# Autodesk Inventor assembly: ControlBox
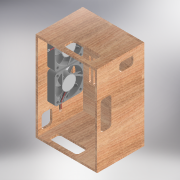
[picture p0: Inventor's stored thumbnail of the model, 180x180]
Saved by Autodesk Inventor 2018.2 (Build 222227000, 227)
## iProperties
Created: 2018-03-27
Part Number: ControlBox
Document SubType Name: Assembly
Designer: mansu
Author: mansu
## Documents named in this file (6)
- C:\Users\Moochster\OneDrive\Documents\2018 UBC\ELEC 391\Controller\cad\release\ControlBox.iam
- C:\Users\Moochster\OneDrive\Documents\2018 UBC\ELEC 391\Controller\cad\release\ControlBoxTop.ipt
- C:\Users\Moochster\OneDrive\Documents\2018 UBC\ELEC 391\Controller\cad\release\ControlBoxFace.ipt
- C:\Users\Moochster\OneDrive\Documents\2018 UBC\ELEC 391\Controller\cad\release\40x40x10 DC Fan.ipt
- C:\Users\Moochster\OneDrive\Documents\2018 UBC\ELEC 391\Controller\cad\release\ControlBoxFlatFace.ipt
- C:\Users\Moochster\OneDrive\Documents\2018 UBC\ELEC 391\Controller\cad\release\ControlBoxSide.ipt
## Components (7 placed, 5 different names)
1. ControlBoxTop:1 — Flush:5, Flush:6, Flush:8, Flush:9
2. ControlBoxFlatFace:1 — Flush:5, Mate:17, Mate:18, Mate:19, Mate:20, Flush:8
3. ControlBoxFace:2 — Flush:6, Mate:12, Mate:13, Mate:14, Mate:15, Mate:16, Mate:21, Mate:22
4. 40x40x10 DC Fan:1 — Mate:12, Flush:7, Mate:14, Mate:15
5. 40x40x10 DC Fan:2 — Mate:13, Flush:7, Mate:16
6. ControlBoxSide:1 — Mate:17, Mate:18, Mate:21, Mate:22, Flush:9
7. ControlBoxSide:2 — Mate:19, Mate:20
## Relationships (16: Mate 11, Flush 5)
- Flush:5: ControlBoxTop:1 ↔ ControlBoxFlatFace:1
- Flush:6: ControlBoxTop:1 ↔ ControlBoxFace:2
- Mate:12: ControlBoxFace:2 ↔ 40x40x10 DC Fan:1
- Mate:13: ControlBoxFace:2 ↔ 40x40x10 DC Fan:2
- Flush:7: 40x40x10 DC Fan:1 ↔ 40x40x10 DC Fan:2
- Mate:14: ControlBoxFace:2 ↔ 40x40x10 DC Fan:1
- Mate:15: ControlBoxFace:2 ↔ 40x40x10 DC Fan:1
- Mate:16: ControlBoxFace:2 ↔ 40x40x10 DC Fan:2
- Mate:17: ControlBoxFlatFace:1 ↔ ControlBoxSide:1
- Mate:18: ControlBoxFlatFace:1 ↔ ControlBoxSide:1
- Mate:19: ControlBoxFlatFace:1 ↔ ControlBoxSide:2
- Mate:20: ControlBoxFlatFace:1 ↔ ControlBoxSide:2
- Mate:21: ControlBoxFace:2 ↔ ControlBoxSide:1
- Mate:22: ControlBoxFace:2 ↔ ControlBoxSide:1
- Flush:8: ControlBoxTop:1 ↔ ControlBoxFlatFace:1
- Flush:9: ControlBoxTop:1 ↔ ControlBoxSide:1
